# Autodesk Inventor assembly: 090 ASY bottom
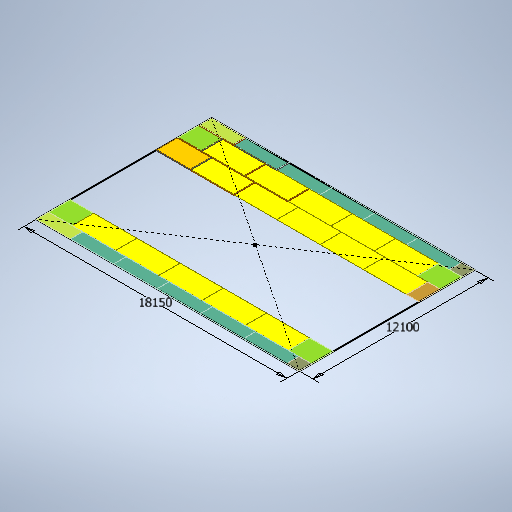
[picture p0: Inventor's stored thumbnail of the model, 512x512]
Saved by Autodesk Inventor 2026.2 (Build 302298000, 298)
## iProperties
Created: 2026-05-19
Part Number: 090 ASY bottom
Document SubType Name: Assembly
Designer: user
Author: user
## Documents named in this file (14)
- C:\Users\admin\Documents\Inventor\GBK-Gubkinskiy\090 ASY bottom.iam
- C:\Users\admin\Documents\Inventor\GBK-Gubkinskiy\Пол\0921_CPY1.ipt
- C:\Users\admin\Documents\Inventor\GBK-Gubkinskiy\Пол\0922_CPY1.ipt
- C:\Users\admin\Documents\Inventor\GBK-Gubkinskiy\Пол\0923_CPY1.ipt
- C:\Users\admin\Documents\Inventor\GBK-Gubkinskiy\Пол\0931_CPY.ipt
- C:\Users\admin\Documents\Inventor\GBK-Gubkinskiy\Пол\0931_CPY1.ipt
- C:\Users\admin\Documents\Inventor\GBK-Gubkinskiy\Пол\0932_CPY1.ipt
- C:\Users\admin\Documents\Inventor\GBK-Gubkinskiy\Пол\0921_CPY.ipt
- C:\Users\admin\Documents\Inventor\GBK-Gubkinskiy\Пол\0923_CPY.ipt
- C:\Users\admin\Documents\Inventor\GBK-Gubkinskiy\Пол\0921_CPY1_CPY.ipt
- C:\Users\admin\Documents\Inventor\GBK-Gubkinskiy\Пол\GBK bottom 0231.ipt
- C:\Users\admin\Documents\Inventor\GBK-Gubkinskiy\Пол\GBK bottom 0233.ipt
- C:\Users\admin\Documents\Inventor\GBK-Gubkinskiy\ASY GBK bottom 0010.iam
- C:\Users\admin\Documents\Inventor\GBK-Gubkinskiy\Пол\0932_CPY1_CPY.ipt
## Components (43 placed, 13 different names)
1. 0923_CPY:1 — Rigid:43, Mate:13, Mate:14
2. 0932_CPY1:1 — Rigid:43, Mate:15
3. 0931_CPY1:1 — Rigid:21
4. 0921_CPY1:1 — Rigid:13, Mate:2, Mate:3, Rigid:14, Mate:13, Mate:14, Mate:15
5. GBK bottom 0123:1 — Rigid:14, Rigid:17, Mate:7, Mate:8, Mate:9
6. GBK bottom 0123:2 — Rigid:17, Rigid:18
7. GBK bottom 0123:3 — Rigid:18, Rigid:19
8. GBK bottom 0123:4 — Rigid:19, Rigid:20
9. GBK bottom 0123:5 — Rigid:20, Rigid:21
10. 0931_CPY:3 — Rigid:36
11. 0921_CPY:11
12. 0921_CPY:12
13. 0921_CPY:13
14. 0921_CPY:14
15. 0921_CPY:15
16. 0931_CPY:4
17. 0921_CPY1:2 — Rigid:36
18. 0931_CPY1:2
19. GBK bottom 0123:6
20. GBK bottom 0123:7
21. GBK bottom 0123:8
22. GBK bottom 0123:9
23. GBK bottom 0123:10
24. 0922_CPY1:4 — Rigid:42, Mate:8
25. 0923_CPY:2 — Rigid:42, Mate:7, Mate:9
26. 0923_CPY1:1 — Mate:5, Rigid:41
27. GBK bottom 0231:1 — Rigid:15, Rigid:39, Mate:10, Mate:11, Mate:12
28. GBK bottom 0233:1 — Rigid:22
29. 0931_CPY:2 — Rigid:7
30. 0921_CPY:10 — Rigid:22
31. 0921_CPY:5 — Rigid:6, Rigid:7
32. 0921_CPY:9
33. 0921_CPY:4 — Rigid:5, Rigid:6
34. 0921_CPY:8
35. 0921_CPY:3 — Rigid:5, Rigid:38
36. 0921_CPY:7 — Rigid:40
37. ASY GBK bottom 0010:3 [sub-assembly] — Rigid:39, Rigid:40
38. ASY GBK bottom 0010:2 [sub-assembly] — Rigid:37, Rigid:38
39. 0932_CPY1:2 — Rigid:44, Mate:12
40. 0923_CPY1:2 — Rigid:44, Mate:10, Mate:11
41. GBK 0214  bottom:1 — Mate:4, Rigid:41, Mate:6
42. ASY GBK bottom 0010:1 [sub-assembly] — Rigid:37
43. 0931_CPY:1 — Mate:1, Rigid:13, Rigid:15, Mate:4, Mate:5, Mate:6
## Relationships (52: WeldJoint 37, Mate 15)
- [WeldJoint] (4 mm): ASY GBK bottom 0010:1 ↔ 0931_CPY:1
- Rigid:5 [WeldJoint] (4 mm): 0921_CPY:4 ↔ 0921_CPY:3
- Rigid:6 [WeldJoint] (4 mm): 0921_CPY:5 ↔ 0921_CPY:4
- Rigid:7 [WeldJoint] (4 mm): 0931_CPY:2 ↔ 0921_CPY:5
- Mate:1 (-9075 mm): 0931_CPY:1
- [WeldJoint] (4 mm): 0921_CPY:8 ↔ 0921_CPY:7
- [WeldJoint] (4 mm): 0921_CPY:9 ↔ 0921_CPY:8
- [WeldJoint] (4 mm): 0921_CPY:10 ↔ 0921_CPY:9
- Rigid:13 [WeldJoint] (4 mm): 0921_CPY1:1 ↔ 0931_CPY:1
- Mate:2: 0921_CPY1:1
- Mate:3 (-6050 mm): 0921_CPY1:1
- Rigid:14 [WeldJoint] (4 mm): 0921_CPY1:1 ↔ GBK bottom 0123:1
- Rigid:15 [WeldJoint] (4 mm): GBK bottom 0231:1 ↔ 0931_CPY:1
- Rigid:17 [WeldJoint] (4 mm): GBK bottom 0123:1 ↔ GBK bottom 0123:2
- Rigid:18 [WeldJoint] (4 mm): GBK bottom 0123:2 ↔ GBK bottom 0123:3
- Rigid:19 [WeldJoint] (4 mm): GBK bottom 0123:3 ↔ GBK bottom 0123:4
- Rigid:20 [WeldJoint] (4 mm): GBK bottom 0123:4 ↔ GBK bottom 0123:5
- Rigid:21 [WeldJoint] (4 mm): 0931_CPY1:1 ↔ GBK bottom 0123:5
- Rigid:22 [WeldJoint] (4 mm): GBK bottom 0233:1 ↔ 0921_CPY:10
- [WeldJoint] (4 mm): 0931_CPY:3 ↔ 0921_CPY:11
- [WeldJoint] (4 mm): 0921_CPY:11 ↔ 0921_CPY:12
- [WeldJoint] (4 mm): 0921_CPY:12 ↔ 0921_CPY:13
- [WeldJoint] (4 mm): 0921_CPY:13 ↔ 0921_CPY:14
- [WeldJoint] (4 mm): 0921_CPY:14 ↔ 0921_CPY:15
- [WeldJoint] (4 mm): 0921_CPY:15 ↔ 0931_CPY:4
- [WeldJoint] (4 mm): 0921_CPY1:2 ↔ GBK bottom 0123:6
- [WeldJoint] (4 mm): GBK bottom 0123:6 ↔ GBK bottom 0123:7
- [WeldJoint] (4 mm): GBK bottom 0123:7 ↔ GBK bottom 0123:8
- [WeldJoint] (4 mm): GBK bottom 0123:8 ↔ GBK bottom 0123:9
- [WeldJoint] (4 mm): GBK bottom 0123:9 ↔ GBK bottom 0123:10
- [WeldJoint] (4 mm): 0931_CPY1:2 ↔ GBK bottom 0123:10
- Rigid:36 [WeldJoint] (4 mm): 0931_CPY:3 ↔ 0921_CPY1:2
- Rigid:37 [WeldJoint] (4 mm): ASY GBK bottom 0010:2 ↔ ASY GBK bottom 0010:1
- Rigid:38 [WeldJoint] (4 mm): 0921_CPY:3 ↔ ASY GBK bottom 0010:2
- Rigid:39 [WeldJoint] (4 mm): GBK bottom 0231:1 ↔ ASY GBK bottom 0010:3
- Rigid:40 [WeldJoint] (4 mm): 0921_CPY:7 ↔ ASY GBK bottom 0010:3
- Mate:4: GBK 0214  bottom:1 ↔ 0931_CPY:1
- Mate:5 (-30 mm): 0923_CPY1:1 ↔ 0931_CPY:1
- Rigid:41 [WeldJoint]: 0923_CPY1:1 ↔ GBK 0214  bottom:1
- Mate:6 (-30 mm): GBK 0214  bottom:1 ↔ 0931_CPY:1
- Rigid:42 [WeldJoint]: 0922_CPY1:4 ↔ 0923_CPY:2
- Rigid:43 [WeldJoint]: 0923_CPY:1 ↔ 0932_CPY1:1
- Rigid:44 [WeldJoint]: 0932_CPY1:2 ↔ 0923_CPY1:2
- Mate:7: GBK bottom 0123:1 ↔ 0923_CPY:2
- Mate:8 (-30 mm): GBK bottom 0123:1 ↔ 0922_CPY1:4
- Mate:9 (-30 mm): GBK bottom 0123:1 ↔ 0923_CPY:2
- Mate:10: GBK bottom 0231:1 ↔ 0923_CPY1:2
- Mate:11 (-30 mm): GBK bottom 0231:1 ↔ 0923_CPY1:2
- Mate:12 (-30 mm): GBK bottom 0231:1 ↔ 0932_CPY1:2
- Mate:13: 0923_CPY:1 ↔ 0921_CPY1:1
- Mate:14 (-30 mm): 0923_CPY:1 ↔ 0921_CPY1:1
- Mate:15 (-30 mm): 0932_CPY1:1 ↔ 0921_CPY1:1
## Named parameters: d65_d59 = 4 mm, d66_d60 = 4 mm, d67_d61 = 4 mm, d85_d37 = 4 mm, d86_d58 = 4 mm, d87_d59 = 4 mm, d88_d60 = 4 mm, d89_d61 = 4 mm, d90_d62 = 4 mm, d96_d76 = 4 mm, d97_d79 = 4 mm, d98_d80 = 4 mm, d99_d81 = 4 mm, d100_d82 = 4 mm, d101_d83 = 4 mm
